# Autodesk Inventor assembly: Rotule_M2
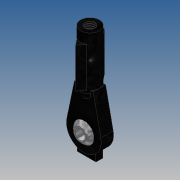
[picture p0: Inventor's stored thumbnail of the model, 180x180]
Saved by Autodesk Inventor 2021.3 (Build 253353000, 353)
## iProperties
Created: 2023-08-17
Part Number: Rotule_M2
Document SubType Name: Assembly
Designer: cedric.clivaz
Author: cedric.clivaz
## Documents named in this file (3)
- I:\Bachelor\SI\Cours\214_SS1\1 - Infos Générales et documentation\_Modele_Structure_dossiers\0 - Structure_R-SYND-SS1_214\1 - Infos Etudiants\1 - CAD Parts\Rotules\Rotule_M2.iam
- I:\Bachelor\SI\Cours\214_SS1\1 - Infos Générales et documentation\_Modele_Structure_dossiers\0 - Structure_R-SYND-SS1_214\1 - Infos Etudiants\1 - CAD Parts\Rotules\Boule_Rotule_M2.ipt
- I:\Bachelor\SI\Cours\214_SS1\1 - Infos Générales et documentation\_Modele_Structure_dossiers\0 - Structure_R-SYND-SS1_214\1 - Infos Etudiants\1 - CAD Parts\Rotules\Rotule_M2.ipt
## Components (2 placed, 2 different names)
1. Boule_Rotule_M2:1 — Tangent:1
2. Rotule_M2:1 — Tangent:1
## Relationships (1: Tangent 1)
- Tangent:1: Boule_Rotule_M2:1 ↔ Rotule_M2:1
